# Autodesk Inventor assembly: B_Legs0_MIR
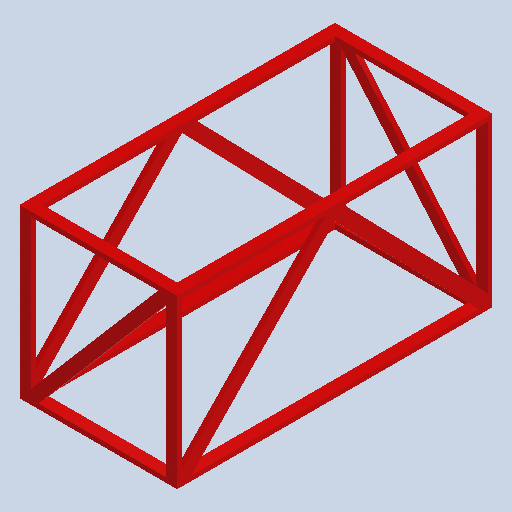
[picture p0: Inventor's stored thumbnail of the model, 512x512]
Saved by Autodesk Inventor 2025 (Build 290162000, 162)
## iProperties
Created: 2024-09-19
Part Number: B_Legs0_MIR
Document SubType Name: Assembly
Designer: localadmin
Author: User
## Documents named in this file (6)
- C:\Users\localadmin\Documents\USCTigerBurn24\Tburn24\Legs0\B_Legs0_MIR.iam
- C:\Users\localadmin\Documents\USCTigerBurn24\Tburn24\Legs0\8'x2x4_MIR.ipt
- C:\Users\localadmin\Documents\USCTigerBurn24\Tburn24\Legs0\3'5x2x4_MIR.ipt
- C:\Users\localadmin\Documents\USCTigerBurn24\Tburn24\Legs0\4x2x4_MIR.ipt
- C:\Users\localadmin\Documents\USCTigerBurn24\Tburn24\Legs0\48x2x4-2_MIR.ipt
- C:\Users\localadmin\Documents\USCTigerBurn24\Tburn24\Legs0\44x2x4_MIR.ipt
## Components (16 placed, 5 different names)
1. 8'x2x4_MIR:1 — Flush:3, Flush:2, Flush:1, Flush:5, Flush:4, Flush:14, Flush:13, Flush:8, Flush:12, Flush:10, Mate:3
2. 8'x2x4_MIR:2 — Flush:3, Flush:2, Flush:1, Mate:1, Flush:7, Flush:6, Mate:2, Flush:16, Flush:15, Mate:5, Flush:11, Flush:9
3. 3'5x2x4_MIR:1 — Flush:5, Flush:4
4. 3'5x2x4_MIR:2 — Flush:7, Flush:6, Mate:2, Mate:4
5. 4x2x4_MIR:1 — Flush:14, Flush:13, Flush:8, Flush:20, Flush:17, Mate:7
6. 4x2x4_MIR:2 — Flush:16, Flush:15, Mate:5, Flush:19, Flush:18, Mate:6, Flush:27
7. 4x2x4_MIR:3 — Flush:11, Flush:9, Mate:4, Mate:11
8. 4x2x4_MIR:4 — Flush:12, Flush:10, Mate:3, Flush:28, Mate:13
9. 8'x2x4_MIR:3 — Flush:20, Flush:17, Mate:7, Mate:8, Flush:24, Flush:23, Mate:9, Flush:25
10. 8'x2x4_MIR:4 — Flush:19, Flush:18, Mate:6, Flush:22, Flush:21, Mate:10, Flush:26
11. 3'5x2x4_MIR:3 — Flush:22, Flush:21, Mate:8, Mate:12
12. 3'5x2x4_MIR:4 — Flush:24, Flush:23, Mate:9
13. 48x2x4-2_MIR:1 — Flush:25
14. 48x2x4-2_MIR:2 — Mate:11, Mate:10, Flush:26
15. 44x2x4_MIR:1 — Flush:27
16. 44x2x4_MIR:2 — Flush:28, Mate:13, Mate:12
## Relationships (41: Flush 23, Mate 18)
- Flush:3: 8'x2x4_MIR:1 ↔ 8'x2x4_MIR:2
- Flush:2 (1130.3 mm): 8'x2x4_MIR:1 ↔ 8'x2x4_MIR:2
- Flush:1: 8'x2x4_MIR:1 ↔ 8'x2x4_MIR:2
- Mate:1: 8'x2x4_MIR:2
- Flush:5 [Mate]: 8'x2x4_MIR:1 ↔ 3'5x2x4_MIR:1
- Flush:4 [Mate]: 8'x2x4_MIR:1 ↔ 3'5x2x4_MIR:1
- Flush:7: 8'x2x4_MIR:2 ↔ 3'5x2x4_MIR:2
- Flush:6: 8'x2x4_MIR:2 ↔ 3'5x2x4_MIR:2
- Mate:2: 8'x2x4_MIR:2 ↔ 3'5x2x4_MIR:2
- Flush:14: 8'x2x4_MIR:1 ↔ 4x2x4_MIR:1
- Flush:13: 8'x2x4_MIR:1 ↔ 4x2x4_MIR:1
- Flush:8 [Mate]: 8'x2x4_MIR:1 ↔ 4x2x4_MIR:1
- Flush:16: 8'x2x4_MIR:2 ↔ 4x2x4_MIR:2
- Flush:15: 8'x2x4_MIR:2 ↔ 4x2x4_MIR:2
- Mate:5: 8'x2x4_MIR:2 ↔ 4x2x4_MIR:2
- Flush:11: 8'x2x4_MIR:2 ↔ 4x2x4_MIR:3
- Flush:9: 8'x2x4_MIR:2 ↔ 4x2x4_MIR:3
- Mate:4: 3'5x2x4_MIR:2 ↔ 4x2x4_MIR:3
- Flush:12: 8'x2x4_MIR:1 ↔ 4x2x4_MIR:4
- Flush:10: 8'x2x4_MIR:1 ↔ 4x2x4_MIR:4
- Mate:3: 8'x2x4_MIR:1 ↔ 4x2x4_MIR:4
- Flush:20: 4x2x4_MIR:1 ↔ 8'x2x4_MIR:3
- Flush:17: 4x2x4_MIR:1 ↔ 8'x2x4_MIR:3
- Mate:7: 4x2x4_MIR:1 ↔ 8'x2x4_MIR:3
- Flush:19: 4x2x4_MIR:2 ↔ 8'x2x4_MIR:4
- Flush:18: 4x2x4_MIR:2 ↔ 8'x2x4_MIR:4
- Mate:6: 4x2x4_MIR:2 ↔ 8'x2x4_MIR:4
- Flush:22: 8'x2x4_MIR:4 ↔ 3'5x2x4_MIR:3
- Flush:21: 8'x2x4_MIR:4 ↔ 3'5x2x4_MIR:3
- Mate:8: 8'x2x4_MIR:3 ↔ 3'5x2x4_MIR:3
- Flush:24: 8'x2x4_MIR:3 ↔ 3'5x2x4_MIR:4
- Flush:23: 8'x2x4_MIR:3 ↔ 3'5x2x4_MIR:4
- Mate:9: 8'x2x4_MIR:3 ↔ 3'5x2x4_MIR:4
- Flush:25 [Mate]: 8'x2x4_MIR:3 ↔ 48x2x4-2_MIR:1
- Mate:11: 4x2x4_MIR:3 ↔ 48x2x4-2_MIR:2
- Mate:10: 8'x2x4_MIR:4 ↔ 48x2x4-2_MIR:2
- Flush:26: 8'x2x4_MIR:4 ↔ 48x2x4-2_MIR:2
- Flush:27 [Mate]: 4x2x4_MIR:2 ↔ 44x2x4_MIR:1
- Flush:28: 4x2x4_MIR:4 ↔ 44x2x4_MIR:2
- Mate:13: 4x2x4_MIR:4 ↔ 44x2x4_MIR:2
- Mate:12: 3'5x2x4_MIR:3 ↔ 44x2x4_MIR:2
